# Autodesk Inventor assembly: s-assy-j3
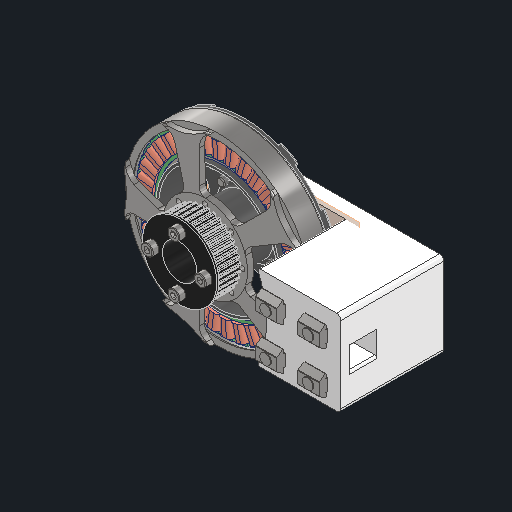
[picture p0: Inventor's stored thumbnail of the model, 512x512]
Saved by Autodesk Inventor 2022 (Build 260153000, 153)
## iProperties
Created: 2021-10-17
Part Number: s-assy-j3
Document SubType Name: Assembly
Designer: Yuta Kage
Mass: 407.494 g
Surface Area: 911.61 cm^2
Volume: 147.16 cm^3
Density: 2.76905 g/cm^3
Author: Yuta Kage
## Documents named in this file (14)
- C:\Users\yuta0\Documents\GitHub\catchrobo_hardware\assy-scara\s-assy-j3.iam
- C:\Users\yuta0\Documents\GitHub\catchrobo_hardware\assy-scara\scara-base22.ipt
- C:\Users\yuta0\Documents\GitHub\catchrobo_hardware\assy-scara\MR148ZZ.ipt
- C:\Users\yuta0\Documents\GitHub\catchrobo_hardware\assy-scara\CB3-15.ipt
- C:\Users\yuta0\Documents\GitHub\catchrobo_hardware\assy-scara\base12.ipt
- C:\Users\yuta0\Documents\GitHub\catchrobo_hardware\assy-scara\ex8108.iam
- C:\Users\yuta0\Documents\GitHub\catchrobo_hardware\assy-scara\CB5-55.ipt
- C:\Users\yuta0\Documents\GitHub\catchrobo_hardware\assy-scara\HNTT5-5.ipt
- C:\Users\yuta0\Documents\GitHub\catchrobo_hardware\assy-scara\CB2-4.ipt
- C:\Users\yuta0\Documents\GitHub\catchrobo_hardware\assy-scara\s-assy-AS5047P-TS_EK_AB.iam
- C:\Users\yuta0\Documents\GitHub\catchrobo_hardware\assy-scara\SB-203040.ipt
- C:\Users\yuta0\Documents\GitHub\catchrobo_hardware\assy-scara\s-assy-scara-magnet.iam
- C:\Users\yuta0\Documents\GitHub\catchrobo_hardware\assy-scara\CB4-10.ipt
- C:\Users\yuta0\Documents\GitHub\catchrobo_hardware\assy-scara\WSJ-STN-M5.ipt
## Components (42 placed, 13 different names)
1. scara-base22:1 — メイト:1, メイト:2, メイト:3, メイト:4, メイト:5, メイト:11, メイト:14, 角度:1, メイト:20, フラッシュ:1, メイト:22, メイト:23, メイト:24, メイト:25, メイト:26, メイト:27, メイト:29
2. base12:1 — メイト:6, メイト:7, メイト:8, メイト:9, メイト:10
3. ex8108:1 [sub-assembly] — メイト:3, メイト:4, メイト:5, メイト:6, メイト:7, メイト:10, メイト:17, メイト:18, メイト:19
4. s-assy-AS5047P-TS_EK_AB:1 [sub-assembly] — メイト:22, メイト:23
5. s-assy-scara-magnet:1 [sub-assembly] — メイト:17, メイト:18, メイト:19
6. MR148ZZ:1 — メイト:1, メイト:2
7. MR148ZZ:2
8. MR148ZZ:3
9. MR148ZZ:4
10. MR148ZZ:5
11. MR148ZZ:6
12. CB3-15:1 — メイト:8, メイト:9
13. CB3-15:2
14. CB3-15:3
15. CB3-15:4
16. CB5-55:1 — メイト:11, メイト:13, メイト:28, メイト:30
17. HNTT5-5:1 — メイト:13, メイト:14, 角度:1
18. WSJ-STN-M5:1 — メイト:28, メイト:29, メイト:30
19. CB5-55:2
20. HNTT5-5:2
21. WSJ-STN-M5:2
22. CB5-55:3
23. HNTT5-5:3
24. WSJ-STN-M5:3
25. CB5-55:4
26. HNTT5-5:4
27. WSJ-STN-M5:4
28. CB2-4:1 — メイト:21
29. SB-203040:1 — メイト:20, フラッシュ:1, メイト:21
30. CB2-4:2
31. SB-203040:2
32. CB2-4:3
33. SB-203040:3
34. CB2-4:4
35. SB-203040:4
36. CB4-10:1 — メイト:24, メイト:25
37. CB4-10:2
38. CB4-10:3
39. CB4-10:4
40. CB3-15:5 — メイト:26, メイト:27
41. CB3-15:6
42. CB3-15:7
## Component patterns: (6 elements, first: MR148ZZ:1), (4 elements, first: CB3-15:1), (4 elements, first: CB5-55:1 + HNTT5-5:1 + WSJ-STN-M5:1), (4 elements, first: CB2-4:1 + SB-203040:1), (4 elements, first: CB4-10:1), (3 elements, first: CB3-15:5)
## Relationships (31: Mate 29, Angle 1, Flush 1)
- メイト:1 [Mate]: scara-base22:1 ↔ MR148ZZ:1
- メイト:2 [Mate]: scara-base22:1 ↔ MR148ZZ:1
- メイト:3 [Mate]: scara-base22:1 ↔ ex8108:1
- メイト:4 [Mate]: scara-base22:1 ↔ ex8108:1
- メイト:5 [Mate]: scara-base22:1 ↔ ex8108:1
- メイト:6 [Mate]: base12:1 ↔ ex8108:1
- メイト:7 [Mate]: base12:1 ↔ ex8108:1
- メイト:8 [Mate]: base12:1 ↔ CB3-15:1
- メイト:9 [Mate]: base12:1 ↔ CB3-15:1
- メイト:10 [Mate]: base12:1 ↔ ex8108:1
- メイト:11 [Mate]: scara-base22:1 ↔ CB5-55:1
- メイト:13 [Mate]: CB5-55:1 ↔ HNTT5-5:1
- メイト:14 [Mate] (2 mm): scara-base22:1 ↔ HNTT5-5:1
- 角度:1 [Angle] (0 deg): scara-base22:1 ↔ HNTT5-5:1
- [Mate]: s-assy-AS5047P-TS_EK_AB:1 ↔ CB2-4:1
- [Mate]: s-assy-AS5047P-TS_EK_AB:1 ↔ CB2-4:1
- メイト:17 [Mate]: ex8108:1 ↔ s-assy-scara-magnet:1
- メイト:18 [Mate]: ex8108:1 ↔ s-assy-scara-magnet:1
- メイト:19 [Mate]: ex8108:1 ↔ s-assy-scara-magnet:1
- メイト:20 [Mate]: scara-base22:1 ↔ SB-203040:1
- フラッシュ:1 [Flush]: scara-base22:1 ↔ SB-203040:1
- メイト:21 [Mate]: CB2-4:1 ↔ SB-203040:1
- メイト:22 [Mate]: scara-base22:1 ↔ s-assy-AS5047P-TS_EK_AB:1
- メイト:23 [Mate]: scara-base22:1 ↔ s-assy-AS5047P-TS_EK_AB:1
- メイト:24 [Mate]: scara-base22:1 ↔ CB4-10:1
- メイト:25 [Mate]: scara-base22:1 ↔ CB4-10:1
- メイト:26 [Mate]: scara-base22:1 ↔ CB3-15:5
- メイト:27 [Mate]: scara-base22:1 ↔ CB3-15:5
- メイト:28 [Mate]: CB5-55:1 ↔ WSJ-STN-M5:1
- メイト:29 [Mate]: scara-base22:1 ↔ WSJ-STN-M5:1
- メイト:30 [Mate]: CB5-55:1 ↔ WSJ-STN-M5:1
